# Autodesk Inventor assembly: 5_left_Arm_joint
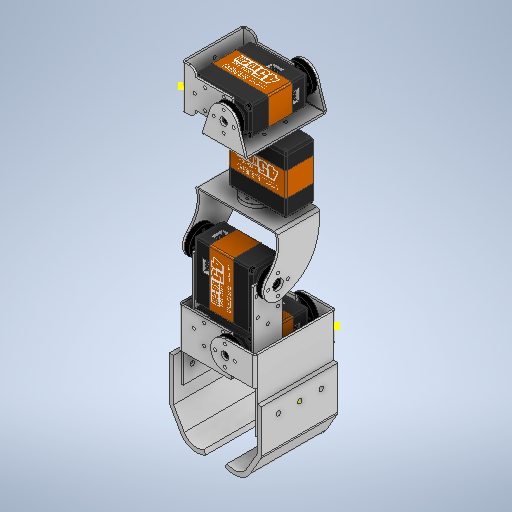
[picture p0: Inventor's stored thumbnail of the model, 512x512]
Saved by Autodesk Inventor 2026.1 (Build 301233020, 233B)
## iProperties
Created: 2026-01-04
Part Number: 5_left_Arm_joint
Document SubType Name: Assembly
Designer: aa992
Author: aa992
## Documents named in this file (13)
- C:\Users\aa992\OneDrive\Desktop\RHp_Humanoid_ver1\Assembly\5_left_Arm_joint.iam
- C:\Users\aa992\OneDrive\Desktop\RHp_Humanoid_ver1\Part\Frame\Arm\axis_13_top_frame.ipt
- C:\Users\aa992\OneDrive\Desktop\RHp_Humanoid_ver1\Part\HTD-45H, Horn\HTD-45H\HTD-45H.iam
- C:\Users\aa992\OneDrive\Desktop\RHp_Humanoid_ver1\Part\HTD-45H, Horn\Horn\Top Horn.ipt
- C:\Users\aa992\OneDrive\Desktop\RHp_Humanoid_ver1\Part\HTD-45H, Horn\Horn\Bottom Horn.ipt
- C:\Users\aa992\OneDrive\Desktop\RHp_Humanoid_ver1\Part\Frame\Arm\axis_14_bottom_frame.ipt
- C:\Users\aa992\OneDrive\Desktop\RHp_Humanoid_ver1\Part\HTD-45H, Horn\Horn\Top Horn silver.ipt
- C:\Users\aa992\OneDrive\Desktop\RHp_Humanoid_ver1\Part\Frame\Arm\axis_15_bottom_frame.ipt
- C:\Users\aa992\OneDrive\Desktop\RHp_Humanoid_ver1\Part\Frame\Arm\axis_16_top_frame.ipt
- C:\Users\aa992\OneDrive\Desktop\RHp_Humanoid_ver1\Part\Frame\Arm\axis_16_bottom_frame.ipt
- C:\Users\aa992\OneDrive\Desktop\RHp_Humanoid_ver1\Part\Frame\Arm\axis_17_top_frame.ipt
- C:\Users\aa992\OneDrive\Desktop\RHp_Humanoid_ver1\Part\Frame\Arm\axis_17_bottom_frame.ipt
- C:\Users\aa992\OneDrive\Desktop\RHp_Humanoid_ver1\Part\Frame\Arm\gripper_frame.ipt
## Components (20 placed, 12 different names)
1. axis_13_top_frame:1 — Mate:1, Flush:1, Flush:2, Rigid:1
2. HTD-45H:1 [sub-assembly] — Rigid:1, Rotational:1, Rigid:2
3. Top Horn:1 — Rotational:1
4. Bottom Horn:1 — Rigid:2, Rigid:3
5. axis_14_bottom_frame:1 — Rigid:3, Rigid:4
6. HTD-45H:2 [sub-assembly] — Rigid:4, Rotational:2
7. Top Horn silver:1 — Rotational:2, Rigid:5
8. axis_15_bottom_frame:1 — Rigid:5, Rigid:9, Rigid:10
9. Top Horn:2 — Rotational:3, Rigid:10
10. Bottom Horn:2 — Rigid:9
11. HTD-45H:3 [sub-assembly] — Rotational:3, Rigid:8
12. axis_16_top_frame:1 — Rigid:8, Rigid:11
13. axis_16_bottom_frame:1 — Rigid:11, Rigid:12, Rigid:14
14. HTD-45H:4 [sub-assembly] — Rigid:12, Rotational:4, Rigid:13
15. Top Horn:3 — Rotational:4, Rigid:15
16. Bottom Horn:3 — Rigid:13
17. axis_17_top_frame:1 — Rigid:14, Rigid:16
18. axis_17_bottom_frame:1 — Rigid:15, Rigid:17
19. gripper_frame:1 — Rigid:16
20. gripper_frame:2 — Rigid:17
## Relationships (22: WeldJoint 15, RevoluteJoint 4, Flush 2, Mate 1)
- Mate:1: axis_13_top_frame:1
- Flush:1: axis_13_top_frame:1
- Flush:2: axis_13_top_frame:1
- Rigid:1 [WeldJoint]: axis_13_top_frame:1 ↔ HTD-45H:1
- Rotational:1 [RevoluteJoint]: HTD-45H:1 ↔ Top Horn:1
- Rigid:2 [WeldJoint]: HTD-45H:1 ↔ Bottom Horn:1
- Rigid:3 [WeldJoint]: Bottom Horn:1 ↔ axis_14_bottom_frame:1
- Rigid:4 [WeldJoint]: axis_14_bottom_frame:1 ↔ HTD-45H:2
- Rotational:2 [RevoluteJoint]: HTD-45H:2 ↔ Top Horn silver:1
- Rigid:5 [WeldJoint]: Top Horn silver:1 ↔ axis_15_bottom_frame:1
- Rotational:3 [RevoluteJoint]: Top Horn:2 ↔ HTD-45H:3
- Rigid:8 [WeldJoint]: HTD-45H:3 ↔ axis_16_top_frame:1
- Rigid:9 [WeldJoint]: axis_15_bottom_frame:1 ↔ Bottom Horn:2
- Rigid:10 [WeldJoint]: axis_15_bottom_frame:1 ↔ Top Horn:2
- Rigid:11 [WeldJoint]: axis_16_top_frame:1 ↔ axis_16_bottom_frame:1
- Rigid:12 [WeldJoint]: axis_16_bottom_frame:1 ↔ HTD-45H:4
- Rotational:4 [RevoluteJoint]: HTD-45H:4 ↔ Top Horn:3
- Rigid:13 [WeldJoint]: HTD-45H:4 ↔ Bottom Horn:3
- Rigid:14 [WeldJoint]: axis_16_bottom_frame:1 ↔ axis_17_top_frame:1
- Rigid:15 [WeldJoint]: Top Horn:3 ↔ axis_17_bottom_frame:1
- Rigid:16 [WeldJoint]: axis_17_top_frame:1 ↔ gripper_frame:1
- Rigid:17 [WeldJoint]: axis_17_bottom_frame:1 ↔ gripper_frame:2
